# Autodesk Inventor assembly: High Strength 36-Tooth Gear-With Free Spinning Gear Insert
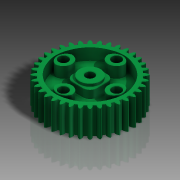
[picture p0: Inventor's stored thumbnail of the model, 180x180]
Saved by Autodesk Inventor 2011 (Build 150239000, 239)
## iProperties
Created: 2010-10-31
Part Number: High Strength 36-Tooth Gear-With Free Spinning Gear Insert
Document SubType Name: Assembly
Designer: JordanK
Author: JordanK
## Documents named in this file (3)
- C:\Users\Public\Documents\Vex CAD Parts\Gears & Pulleys\High Strength 36-Tooth Gear-With Free Spinning Gear Insert.iam
- C:\Users\Public\Documents\Vex CAD Parts\Gears & Pulleys\High Strength 36-Tooth Gear.ipt
- C:\Users\Public\Documents\Vex CAD Parts\Gears & Pulleys\Free Spinning Gear Insert.ipt
## Components (3 placed, 2 different names)
1. High Strength 36-Tooth Gear:1 — Mate:1, Mate:2, Mate:3, Mate:4
2. Free Spinning Gear Insert:1 — Mate:1, Mate:2
3. Free Spinning Gear Insert:2 — Mate:3, Mate:4
## Relationships (4: Mate 4)
- Mate:1: High Strength 36-Tooth Gear:1 ↔ Free Spinning Gear Insert:1
- Mate:2: High Strength 36-Tooth Gear:1 ↔ Free Spinning Gear Insert:1
- Mate:3: High Strength 36-Tooth Gear:1 ↔ Free Spinning Gear Insert:2
- Mate:4: High Strength 36-Tooth Gear:1 ↔ Free Spinning Gear Insert:2
